# Autodesk Inventor assembly: Конвейр сборка
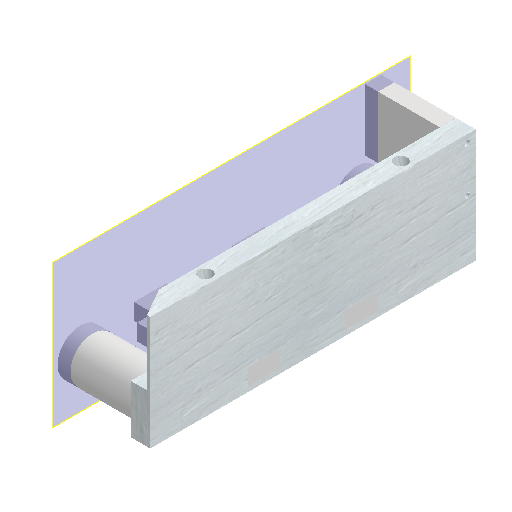
[picture p0: Inventor's stored thumbnail of the model, 512x512]
Saved by Autodesk Inventor 2022 (Build 260153000, 153)
## iProperties
Created: 2023-02-18
Part Number: Конвейр сборка
Document SubType Name: Assembly
Designer: Глеб
Mass: 263.571 g
Surface Area: 706.886 cm^2
Volume: 263.571 cm^3
Density: 1 g/cm^3
Author: Глеб
## Documents named in this file (6)
- C:\Users\Глеб\Documents\Inventor\Файлы Inventor\Конвейр без шпилек сборка.iam
- C:\Users\Глеб\Documents\Inventor\Файлы Inventor\Подставка для двигателя и драйвера.ipt
- C:\Users\Глеб\Documents\Inventor\Файлы Inventor\Вал конвейера.ipt
- C:\Users\Глеб\Documents\Inventor\Файлы Inventor\Вал конвейера 2.ipt
- C:\Users\Глеб\Documents\Inventor\Файлы Inventor\Стенкка для ковнейера.ipt
- C:\Users\Глеб\Documents\Inventor\Файлы Inventor\Стенка конвейера пердняя.ipt
## Components (6 placed, 5 different names)
1. Вал конвейера:1
2. Вал конвейера 2:1
3. Подставка для двигателя и драйвера:2 — Заподлицо:1, Совмещение:29, Совмещение:30
4. Стенкка для ковнейера:1
5. Подставка для двигателя и драйвера:3
6. Стенка конвейера пердняя:1 — Заподлицо:1, Совмещение:29, Совмещение:30
## Relationships (3: Mate 2, Flush 1)
- Заподлицо:1 [Flush]: Подставка для двигателя и драйвера:2 ↔ Стенка конвейера пердняя:1
- Совмещение:29 [Mate]: Подставка для двигателя и драйвера:2 ↔ Стенка конвейера пердняя:1
- Совмещение:30 [Mate]: Подставка для двигателя и драйвера:2 ↔ Стенка конвейера пердняя:1
